# Autodesk Inventor assembly: CHA_006_CenterPulleyAssembly
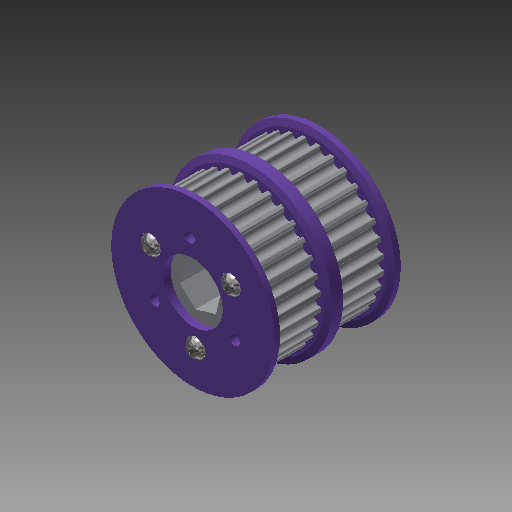
[picture p0: Inventor's stored thumbnail of the model, 512x512]
Saved by Autodesk Inventor 2018 (Build 220112000, 112)
## iProperties
Created: 2020-01-23
Part Number: CHA_006_CenterPulleyAssembly
Document SubType Name: Assembly
Designer: user
Mass: 80.3639 g
Surface Area: 341.88 cm^2
Volume: 73.8125 cm^3
Density: 1.08876 g/cm^3
Author: user
## Documents named in this file (5)
- C:\Users\user\Documents\GrabCAD\New folder\Build season\CHA_006_DrivePulleyAssembly.iam
- C:\Users\user\Documents\GrabCAD\New folder\Build season\CHA_003_DrivePulley.ipt
- C:\Users\user\Documents\GrabCAD\New folder\Build season\CHA_004_DrivePulleyFlange.ipt
- C:\Users\user\Documents\GrabCAD\New folder\Build season\CHA_005_DrivePulleyCenterFlange.ipt
- C:\Users\user\Documents\GrabCAD\New folder\Build season\CHA_008_PulleyScrew(6-32 0.5in)ButtonHeadScrew_MC-91255A148.ipt
## Components (11 placed, 4 different names)
1. CHA_003_DrivePulley:1 — Insert:1, Mate:2, Mate:3
2. CHA_003_DrivePulley:2 — Insert:2, Mate:1, Mate:7, Mate:8
3. CHA_004_DrivePulleyFlange:2 — Insert:2, Mate:1, Mate:6, Insert:6, Insert:7, Insert:8
4. CHA_004_DrivePulleyFlange:3 — Insert:1, Mate:2, Mate:4, Mate:5, Mate:6, Mate:8, Insert:3, Insert:4, Insert:5
5. CHA_005_DrivePulleyCenterFlange:1 — Mate:3, Mate:4, Mate:5, Mate:7
6. CHA_008_PulleyScrew(6-32 0.5in)ButtonHeadScrew_MC-91255A148:1 — Insert:3
7. CHA_008_PulleyScrew(6-32 0.5in)ButtonHeadScrew_MC-91255A148:2 — Insert:7
8. CHA_008_PulleyScrew(6-32 0.5in)ButtonHeadScrew_MC-91255A148:3 — Insert:6
9. CHA_008_PulleyScrew(6-32 0.5in)ButtonHeadScrew_MC-91255A148:4 — Insert:4
10. CHA_008_PulleyScrew(6-32 0.5in)ButtonHeadScrew_MC-91255A148:5 — Insert:8
11. CHA_008_PulleyScrew(6-32 0.5in)ButtonHeadScrew_MC-91255A148:6 — Insert:5
## Relationships (16: Insert 8, Mate 8)
- Insert:1: CHA_003_DrivePulley:1 ↔ CHA_004_DrivePulleyFlange:3
- Insert:2: CHA_003_DrivePulley:2 ↔ CHA_004_DrivePulleyFlange:2
- Mate:1: CHA_003_DrivePulley:2 ↔ CHA_004_DrivePulleyFlange:2
- Mate:2: CHA_003_DrivePulley:1 ↔ CHA_004_DrivePulleyFlange:3
- Mate:3: CHA_003_DrivePulley:1 ↔ CHA_005_DrivePulleyCenterFlange:1
- Mate:4: CHA_004_DrivePulleyFlange:3 ↔ CHA_005_DrivePulleyCenterFlange:1
- Mate:5: CHA_004_DrivePulleyFlange:3 ↔ CHA_005_DrivePulleyCenterFlange:1
- Mate:6: CHA_004_DrivePulleyFlange:2 ↔ CHA_004_DrivePulleyFlange:3
- Mate:7: CHA_003_DrivePulley:2 ↔ CHA_005_DrivePulleyCenterFlange:1
- Mate:8: CHA_003_DrivePulley:2 ↔ CHA_004_DrivePulleyFlange:3
- Insert:3: CHA_004_DrivePulleyFlange:3 ↔ CHA_008_PulleyScrew(6-32 0.5in)ButtonHeadScrew_MC-91255A148:1
- Insert:4: CHA_004_DrivePulleyFlange:3 ↔ CHA_008_PulleyScrew(6-32 0.5in)ButtonHeadScrew_MC-91255A148:4
- Insert:5: CHA_004_DrivePulleyFlange:3 ↔ CHA_008_PulleyScrew(6-32 0.5in)ButtonHeadScrew_MC-91255A148:6
- Insert:6: CHA_004_DrivePulleyFlange:2 ↔ CHA_008_PulleyScrew(6-32 0.5in)ButtonHeadScrew_MC-91255A148:3
- Insert:7: CHA_004_DrivePulleyFlange:2 ↔ CHA_008_PulleyScrew(6-32 0.5in)ButtonHeadScrew_MC-91255A148:2
- Insert:8: CHA_004_DrivePulleyFlange:2 ↔ CHA_008_PulleyScrew(6-32 0.5in)ButtonHeadScrew_MC-91255A148:5
